# Autodesk Inventor assembly: Car Seats
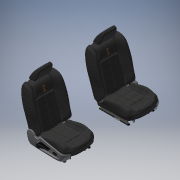
[picture p0: Inventor's stored thumbnail of the model, 180x180]
Saved by Autodesk Inventor 2019 (Build 230136000, 136)
## iProperties
Company: Autodesk Inc.
Created: 2017-07-27
Part Number: Car Seats
Document SubType Name: Assembly
Designer: Autodesk Inc.
Author: Inventor
## Documents named in this file (3)
- C:\Samples\Car Seat\Workspace\Car Seats.iam
- C:\Samples\Car Seat\Workspace\Car Seat.iam
- C:\Samples\Car Seat\Workspace\Car Seat_MIR.iam
## Components (2 placed, 2 different names)
1. Car Seat:1 [sub-assembly] — Flush:1, Flush:2, Flush:3
2. Car Seat_MIR:1 [sub-assembly] — Mate:5, Flush:5, Flush:6
## Relationships (6: Flush 5, Mate 1)
- Flush:1: Car Seat:1
- Flush:2: Car Seat:1
- Flush:3: Car Seat:1
- Mate:5: Car Seat_MIR:1
- Flush:5: Car Seat_MIR:1
- Flush:6: Car Seat_MIR:1
